# Autodesk Inventor assembly: AsemblyV4
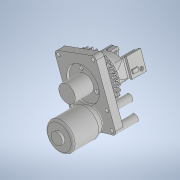
[picture p0: Inventor's stored thumbnail of the model, 180x180]
Saved by Autodesk Inventor 2022 (Build 260153070, 153G)
## iProperties
Created: 2022-01-11
Part Number: AsemblyV4
Document SubType Name: Assembly
Designer: a laptop
Author: a laptop
## Documents named in this file (12)
- C:\Users\a laptop\Desktop\SumoBot\sumobotLIDAR\AssemblyV4\AsemblyV4.iam
- C:\Users\a laptop\Desktop\SumoBot\sumobotLIDAR\AssemblyV4\BASE_PLATE.ipt
- C:\Users\a laptop\Desktop\SumoBot\sumobotLIDAR\AssemblyV4\6703zz.ipt
- C:\Users\a laptop\Desktop\SumoBot\sumobotLIDAR\REF_PART\MOTOR.ipt
- C:\Users\a laptop\Desktop\SumoBot\sumobotLIDAR\REF_PART\SRM-12-06A.ipt
- C:\Users\a laptop\Desktop\SumoBot\sumobotLIDAR\REF_PART\AS5600.ipt
- C:\Users\a laptop\Desktop\SumoBot\sumobotLIDAR\AssemblyV4\VL53LDK.ipt
- C:\Users\a laptop\Desktop\SumoBot\sumobotLIDAR\REF_PART\Magnet.ipt
- C:\Users\a laptop\Desktop\SumoBot\sumobotLIDAR\AssemblyV4\AS5600HolderV2.ipt
- C:\Users\a laptop\Desktop\SumoBot\sumobotLIDAR\AssemblyV4\AsemblyV4\Design Accelerator\Spur Gears1.iam
- C:\Users\a laptop\Desktop\SumoBot\sumobotLIDAR\AssemblyV4\BigGearV8.ipt
- C:\Users\a laptop\Desktop\SumoBot\sumobotLIDAR\AssemblyV4\SmallGearV8.ipt
## Components (12 placed, 11 different names)
1. BASE_PLATE:1 — Mate:31, Mate:34, Mate:35, Mate:38, Mate:41, Mate:42
2. 6703zz:1 — Mate:1, Mate:38, Flush:1
3. SRM-12-06A:1 — Mate:1, Mate:4, Mate:5, Mate:8, Mate:31
4. AS5600:1 — Mate:19, Mate:26, Mate:27, Mate:28, Mate:29
5. VL53LDK:1 — Mate:46, Mate:47, Angle:5
6. VL53LDK:2 — Mate:44, Mate:45, Angle:4
7. Magnet:1 — Mate:26, Mate:43
8. AS5600HolderV2:1 — Mate:27, Mate:28, Mate:29
9. MOTOR:1 — Mate:34, Mate:35, Mate:39, Mate:40, Mate:41
10. Spur Gears:2 [sub-assembly]
11. BigGearV8:1 — Mate:42, Flush:1, Mate:44, Mate:45, Angle:4, Mate:46, Mate:47, Angle:5, Tangent:1, Rotation:1
12. SmallGearV8:1 — Mate:39, Mate:40, Mate:43, Tangent:1, Rotation:1
## Relationships (31: Mate 25, Angle 3, Flush 1, Tangent 1, RelateRotation 1)
- Mate:1: 6703zz:1 ↔ SRM-12-06A:1
- Mate:4: SRM-12-06A:1
- Mate:5: SRM-12-06A:1
- Mate:6
- Mate:7
- Mate:8: SRM-12-06A:1
- Mate:9
- Angle:3 (90 deg)
- Mate:19: AS5600:1
- Mate:26 (0.3 mm): AS5600:1 ↔ Magnet:1
- Mate:27: AS5600:1 ↔ AS5600HolderV2:1
- Mate:28: AS5600:1 ↔ AS5600HolderV2:1
- Mate:29: AS5600:1 ↔ AS5600HolderV2:1
- Mate:31: BASE_PLATE:1 ↔ SRM-12-06A:1
- Mate:34: BASE_PLATE:1 ↔ MOTOR:1
- Mate:35: BASE_PLATE:1 ↔ MOTOR:1
- Mate:38: BASE_PLATE:1 ↔ 6703zz:1
- Mate:39: MOTOR:1 ↔ SmallGearV8:1
- Mate:40: MOTOR:1 ↔ SmallGearV8:1
- Mate:41: BASE_PLATE:1 ↔ MOTOR:1
- Mate:42: BASE_PLATE:1 ↔ BigGearV8:1
- Flush:1: 6703zz:1 ↔ BigGearV8:1
- Mate:43: Magnet:1 ↔ SmallGearV8:1
- Mate:44: VL53LDK:2 ↔ BigGearV8:1
- Mate:45: VL53LDK:2 ↔ BigGearV8:1
- Angle:4 (0 deg): VL53LDK:2 ↔ BigGearV8:1
- Mate:46: VL53LDK:1 ↔ BigGearV8:1
- Mate:47: VL53LDK:1 ↔ BigGearV8:1
- Angle:5 (0 deg): VL53LDK:1 ↔ BigGearV8:1
- Tangent:1: BigGearV8:1 ↔ SmallGearV8:1
- Rotation:1 [RelateRotation] (4.2857 ul): BigGearV8:1 ↔ SmallGearV8:1
